# Autodesk Inventor assembly: Twist Assembly
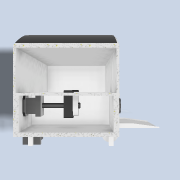
[picture p0: Inventor's stored thumbnail of the model, 180x180]
Saved by Autodesk Inventor 2021 (Build 250183000, 183)
## iProperties
Created: 2021-03-24
Part Number: Twist Assembly
Document SubType Name: Assembly
Designer: calst
Author: calst
## Documents named in this file (7)
- C:\Users\calst\OneDrive\Desktop\University Work\Year 3\Semester 2\Integrated Group Robotics Project\Group Task\AutoDesk Inventor\Servo\Twist Assembly.iam
- C:\Users\calst\OneDrive\Desktop\University Work\Year 3\Semester 2\Integrated Group Robotics Project\Group Task\AutoDesk Inventor\Servo\Gear.ipt
- C:\Users\calst\OneDrive\Desktop\University Work\Year 3\Semester 2\Integrated Group Robotics Project\Group Task\AutoDesk Inventor\Servo\Twist Body.ipt
- C:\Users\calst\OneDrive\Desktop\University Work\Year 3\Semester 2\Integrated Group Robotics Project\Group Task\AutoDesk Inventor\Servo\Shaft.ipt
- C:\Users\calst\OneDrive\Desktop\University Work\Year 3\Semester 2\Integrated Group Robotics Project\Group Task\AutoDesk Inventor\Servo\Motor Shaft.ipt
- C:\Users\calst\OneDrive\Desktop\University Work\Year 3\Semester 2\Integrated Group Robotics Project\Group Task\AutoDesk Inventor\Servo\Servo Motor.ipt
- C:\Users\calst\OneDrive\Desktop\University Work\Year 3\Semester 2\Integrated Group Robotics Project\Group Task\AutoDesk Inventor\Servo\sHUFFLE.ipt
## Components (12 placed, 6 different names)
1. Gear:1 — Rotational:2
2. Gear:2 — Rotational:1
3. Twist Body:1 — Rotational:1, Insert:1, Rotational:2, Insert:2, Insert:7, Insert:8, Mate:2, Insert:10, Insert:11, Mate:3
4. Shaft:1 — Insert:1
5. Motor Shaft:1 — Insert:2, Rotational:3
6. Servo Motor:1 — Rotational:3
7. Motor Shaft:3 — Insert:7, Insert:9
8. sHUFFLE:2 — Insert:11
9. sHUFFLE:3 — Insert:8
10. Servo Motor:4 — Insert:9, Mate:2
11. Servo Motor:5 — Insert:12, Mate:3
12. Motor Shaft:4 — Insert:10, Insert:12
## Relationships (13: Insert 8, RevoluteJoint 3, Mate 2)
- Rotational:1 [RevoluteJoint] (-0.5 mm): Gear:2 ↔ Twist Body:1
- Insert:1: Twist Body:1 ↔ Shaft:1
- Rotational:2 [RevoluteJoint] (-0.5 mm): Gear:1 ↔ Twist Body:1
- Insert:2: Twist Body:1 ↔ Motor Shaft:1
- Rotational:3 [RevoluteJoint]: Motor Shaft:1 ↔ Servo Motor:1
- Insert:7: Twist Body:1 ↔ Motor Shaft:3
- Insert:8: Twist Body:1 ↔ sHUFFLE:3
- Insert:9: Motor Shaft:3 ↔ Servo Motor:4
- Mate:2: Twist Body:1 ↔ Servo Motor:4
- Insert:10: Twist Body:1 ↔ Motor Shaft:4
- Insert:11: Twist Body:1 ↔ sHUFFLE:2
- Insert:12: Servo Motor:5 ↔ Motor Shaft:4
- Mate:3: Twist Body:1 ↔ Servo Motor:5
